# Autodesk Inventor assembly: Hinge
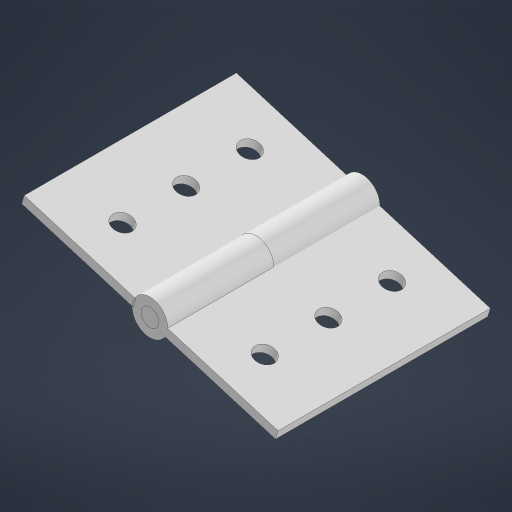
[picture p0: Inventor's stored thumbnail of the model, 512x512]
Saved by Autodesk Inventor 2023 (Build 270158000, 158)
## iProperties
Created: 2021-11-10
Part Number: Hinge
Document SubType Name: Assembly
Designer: 17185
Author: 17185
## Documents named in this file (3)
- C:\Users\seene\Desktop\Stony Brook\SBRT\RoboRescue\GrabCAD\Robocup Rescue\Chassis\Hinge\Hinge.iam
- C:\Users\seene\Desktop\Stony Brook\SBRT\RoboRescue\GrabCAD\Robocup Rescue\Chassis\Hinge\leaf.ipt
- C:\Users\seene\Desktop\Stony Brook\SBRT\RoboRescue\GrabCAD\Robocup Rescue\Chassis\Hinge\Pin.ipt
## Components (3 placed, 2 different names)
1. leaf:1 — Mate:1, Flush:1, Flush:3
2. leaf:2 — Flush:2, Mate:2, Flush:3
3. Pin:1 — Mate:1, Flush:1, Flush:2, Mate:2
## Relationships (5: Flush 3, Mate 2)
- Mate:1: leaf:1 ↔ Pin:1
- Flush:1: leaf:1 ↔ Pin:1
- Flush:2: leaf:2 ↔ Pin:1
- Mate:2: leaf:2 ↔ Pin:1
- Flush:3: leaf:1 ↔ leaf:2
